# Autodesk Inventor assembly: Grid_Of_Piers
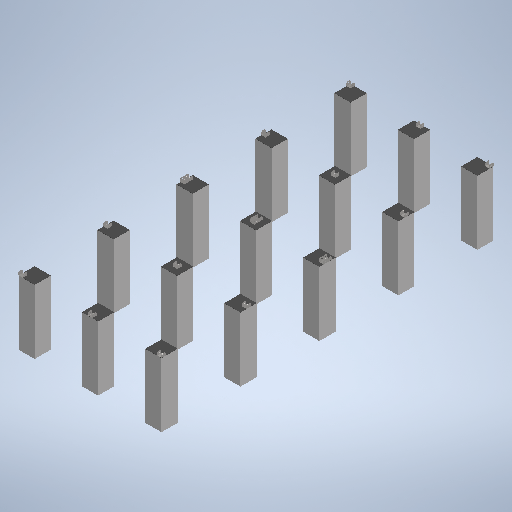
[picture p0: Inventor's stored thumbnail of the model, 512x512]
Saved by Autodesk Inventor 2025 (Build 290162010, 162A)
## iProperties
Created: 2024-08-07
Part Number: Grid_Of_Piers
Document SubType Name: Assembly
Designer: Tom
Author: Tom
## Documents named in this file (7)
- C:\Users\Tom\Documents\Inventor\Mobility\Additional_Building\Area_For_Additional_Buildings_With_Piers\Grid_Of_Piers.iam
- C:\Users\Tom\Documents\Inventor\Mobility\Additional_Building\Area_For_Additional_Buildings_With_Piers\Pier.iam
- C:\Users\Tom\Documents\Inventor\Mobility\Additional_Building\Saddle_Bracket.ipt
- C:\Users\Tom\Documents\Inventor\Mobility\Additional_Building\Saddle_Bracket_MIR.ipt
- C:\Users\Tom\Documents\Inventor\Mobility\Additional_Building\Saddle_Bracket_MIR1.ipt
- C:\Users\Tom\Documents\Inventor\Mobility\Additional_Building\Saddle_Bracket_MIR_MIR.ipt
- C:\Users\Tom\Documents\Inventor\Mobility\Additional_Building\Saddle_Bracket_MIR3.ipt
## Components (33 placed, 6 different names)
1. Saddle_Bracket:1 — Mate:1, Flush:1, Flush:2
2. Saddle_Bracket:2 — Mate:2, Flush:3, Flush:4
3. Saddle_Bracket:3 — Mate:3, Flush:5, Flush:6
4. Saddle_Bracket_MIR:1
5. Saddle_Bracket_MIR:2
6. Saddle_Bracket_MIR:3
7. Saddle_Bracket_MIR1:1
8. Saddle_Bracket_MIR1:2
9. Saddle_Bracket_MIR1:3
10. Saddle_Bracket_MIR_MIR:1
11. Saddle_Bracket_MIR_MIR:2
12. Saddle_Bracket_MIR_MIR:3
13. Saddle_Bracket:4 — Mate:4, Flush:7, Flush:8
14. Saddle_Bracket:5 — Mate:5, Mate:6, Mate:7
15. Saddle_Bracket:6 — Mate:8, Mate:9, Flush:9
16. Saddle_Bracket_MIR3:1
17. Saddle_Bracket_MIR3:2
18. Saddle_Bracket_MIR3:3
19. Pier:1 [sub-assembly] — Mate:1, Flush:1, Flush:2
20. Pier:2 [sub-assembly] — Mate:2, Flush:3, Flush:4
21. Pier:3 [sub-assembly] — Mate:3, Flush:5, Flush:6
22. Pier:4 [sub-assembly]
23. Pier:5 [sub-assembly]
24. Pier:6 [sub-assembly] — Mate:4, Flush:7, Flush:8
25. Pier:7 [sub-assembly] — Mate:5, Mate:6, Mate:7
26. Pier:8 [sub-assembly] — Mate:8, Mate:9, Flush:9
27. Pier:9 [sub-assembly]
28. Pier:10 [sub-assembly]
29. Pier:11 [sub-assembly]
30. Pier:12 [sub-assembly]
31. Pier:13 [sub-assembly]
32. Pier:14 [sub-assembly]
33. Pier:15 [sub-assembly]
## Component patterns: (15 elements, first: Pier:1)
## Relationships (18: Mate 9, Flush 9)
- Mate:1: Saddle_Bracket:1 ↔ Pier:1
- Flush:1 (-3.175 mm): Saddle_Bracket:1 ↔ Pier:1
- Flush:2: Saddle_Bracket:1 ↔ Pier:1
- Mate:2: Saddle_Bracket:2 ↔ Pier:2
- Flush:3 (-3.175 mm): Saddle_Bracket:2 ↔ Pier:2
- Flush:4: Saddle_Bracket:2 ↔ Pier:2
- Mate:3: Saddle_Bracket:3 ↔ Pier:3
- Flush:5 (-3.175 mm): Saddle_Bracket:3 ↔ Pier:3
- Flush:6: Saddle_Bracket:3 ↔ Pier:3
- Mate:4: Saddle_Bracket:4 ↔ Pier:6
- Flush:7: Saddle_Bracket:4 ↔ Pier:6
- Flush:8: Saddle_Bracket:4 ↔ Pier:6
- Mate:5: Saddle_Bracket:5 ↔ Pier:7
- Mate:6: Saddle_Bracket:5 ↔ Pier:7
- Mate:7: Saddle_Bracket:5 ↔ Pier:7
- Mate:8: Saddle_Bracket:6 ↔ Pier:8
- Mate:9: Saddle_Bracket:6 ↔ Pier:8
- Flush:9: Saddle_Bracket:6 ↔ Pier:8
